# Autodesk Inventor assembly: Assembly_v1
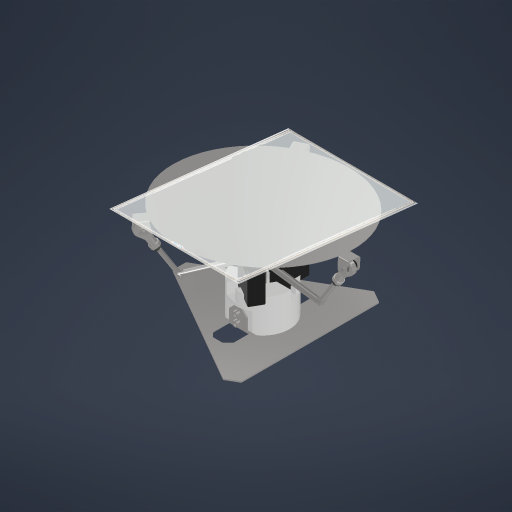
[picture p0: Inventor's stored thumbnail of the model, 512x512]
Saved by Autodesk Inventor 2023 (Build 270158000, 158)
## iProperties
Created: 2023-02-24
Part Number: Assembly_v1
Document SubType Name: Assembly
Designer: roota
Mass: 2034.34 g
Surface Area: 3097.58 cm^2
Volume: 420.227 cm^3
Density: 4.84106 g/cm^3
Author: roota
## Documents named in this file (20)
- D:\GitHub\NTUST-Mechanical-Design\Ball stabilization mechanism\3D CAD files\Mechanical Part CAD files\Assemblies\Assembly_v1.iam
- D:\GitHub\NTUST-Mechanical-Design\Ball stabilization mechanism\3D CAD files\Mechanical Part CAD files\Static Mechanisms\BalancePlate.ipt
- D:\GitHub\NTUST-Mechanical-Design\Ball stabilization mechanism\3D CAD files\Mechanical Part CAD files\Static Mechanisms\BasePlate.ipt
- D:\GitHub\NTUST-Mechanical-Design\Ball stabilization mechanism\3D CAD files\Mechanical Part CAD files\Static Mechanisms\BaseSupport.ipt
- C:\Users\roota\Documents\Inventor\Content Center Files\R2023\en-US\JIS B 2804 E\_JIS B 2804 E - 5 - 6.ipt
- D:\GitHub\NTUST-Mechanical-Design\Ball stabilization mechanism\3D CAD files\Mechanical Part CAD files\Static Mechanisms\rod pin.ipt
- D:\GitHub\NTUST-Mechanical-Design\Ball stabilization mechanism\3D CAD files\Mechanical Part CAD files\Static Mechanisms\4mm spacer.ipt
- D:\GitHub\NTUST-Mechanical-Design\Ball stabilization mechanism\3D CAD files\Mechanical Part CAD files\Hardware Parts\SELF-LUBRIFICATING ROD END\Ball_6mm.ipt
- D:\GitHub\NTUST-Mechanical-Design\Ball stabilization mechanism\3D CAD files\Mechanical Part CAD files\Hardware Parts\SELF-LUBRIFICATING ROD END\End_6mm.ipt
- D:\GitHub\NTUST-Mechanical-Design\Ball stabilization mechanism\3D CAD files\Mechanical Part CAD files\Hardware Parts\M6x1_THREADED_ROD.ipt
- D:\GitHub\NTUST-Mechanical-Design\Ball stabilization mechanism\3D CAD files\Mechanical Part CAD files\Hardware Parts\5mm Bushing.ipt
- D:\GitHub\NTUST-Mechanical-Design\Ball stabilization mechanism\3D CAD files\Mechanical Part CAD files\Dynamic Mechanisms\Servo_Strut.ipt
- C:\Users\roota\Documents\Inventor\Content Center Files\R2023\en-US\ISO 4762(2)\ISO 4762 - M3 x 8ISO.ipt
- D:\GitHub\NTUST-Mechanical-Design\Ball stabilization mechanism\3D CAD files\Mechanical Part CAD files\Hardware Parts\12_1_INCH_TOUCHSCREEN\12inch Touchscreen.ipt
- C:\Users\roota\Documents\Inventor\Content Center Files\R2023\en-US\ISO 4036(2)\ISO 4036 - M6(2).ipt
- C:\Users\roota\Documents\Inventor\Content Center Files\R2023\en-US\ISO 4762(2)\ISO 4762 - M5 x 8ISO.ipt
- D:\GitHub\NTUST-Mechanical-Design\Ball stabilization mechanism\3D CAD files\Electrical Hardware CAD files\SERVO\LDX-335MG_Servo_15kg_cm.ipt
- C:\Users\roota\Documents\Inventor\Content Center Files\R2023\en-US\BS EN ISO 4026\BS EN ISO 4168 - M3 x 6(2).ipt
- D:\GitHub\NTUST-Mechanical-Design\Ball stabilization mechanism\3D CAD files\Mechanical Part CAD files\Static Mechanisms\ServoCap.ipt
- C:\Users\roota\Documents\Inventor\Content Center Files\R2023\en-US\ISO 10642(1)\ISO 10642 - M8 x  60.ipt
## Components (58 placed, 19 different names)
1. BalancePlate:1 — Mate:6, Mate:9, Mate:10, Mate:11, Mate:12, Mate:60, Mate:61, Mate:62, Mate:64, Mate:65, Mate:67, Mate:68, Flush:1, Flush:2, Mate:70, Mate:71, Mate:72, Mate:73, Mate:74, Mate:75, Mate:76, Mate:77, Mate:78, Mate:79, Mate:80, Mate:81, Mate:91, Mate:101
2. BasePlate:1 — Mate:1, Mate:2, Mate:3, Insert:4, Insert:5, Insert:6, Insert:7
3. BaseSupport:1 — Mate:1, Mate:2, Mate:3, Mate:87, Mate:88, Mate:103, Mate:104, Mate:106, Mate:107, Mate:114, Mate:115, Mate:116, Mate:117, Mate:119, Mate:120, Mate:126
4. JIS B 2804 E 5:5 — Mate:5, Mate:8, Mate:10
5. JIS B 2804 E 5:6 — Mate:4, Mate:7
6. rod pin:3 — Mate:4, Mate:5, Mate:6, Mate:7, Mate:8, Mate:9, Mate:13, Mate:14, Mate:15
7. 4mm spacer:1 — Mate:12, Mate:13
8. 4mm spacer:2 — Mate:11, Mate:14, Mate:16
9. Ball_6mm:1 — Mate:15, Mate:16, Mate:17
10. End_6mm:1 — Mate:17, Mate:18, Mate:19, Angle:1, Insert:1
11. M6x1_THREADED_ROD:1 — Mate:18, Mate:19, Mate:20, Mate:23, Angle:1
12. 5mm Bushing:1 — Mate:20, Mate:21, Mate:22, Mate:24
13. Servo_Strut:1 — Mate:21, Mate:22, Mate:23, Mate:25, Mate:85, Mate:86
14. ISO 4762 M3 x 8:1 — Mate:24, Mate:25
15. ISO 4036 M6:1 — Insert:1
16. 12inch Touchscreen:1 — Mate:68, Flush:1, Flush:2
17. JIS B 2804 E 5:7 — Mate:72, Mate:73, Mate:82
18. JIS B 2804 E 5:8 — Mate:62, Mate:74, Mate:75
19. 4mm spacer:5 — Mate:60, Mate:61
20. Ball_6mm:2 — Mate:34, Mate:78, Mate:102
21. End_6mm:2 — Mate:34, Angle:2, Mate:35, Mate:36, Insert:2
22. M6x1_THREADED_ROD:2 — Angle:2, Mate:35, Mate:36, Mate:37, Mate:99
23. 5mm Bushing:2 — Mate:37, Mate:42, Mate:96, Mate:97
24. ISO 4762 M3 x 8:2 — Mate:42, Mate:98
25. ISO 4036 M6:2 — Insert:2
26. JIS B 2804 E 5:10 — Mate:67, Mate:76, Mate:77, Mate:83
27. 4mm spacer:6 — Mate:50, Mate:64, Mate:65
28. Ball_6mm:3 — Mate:50, Mate:51, Mate:79
29. End_6mm:3 — Mate:51, Mate:52, Mate:53, Angle:3, Insert:3
30. M6x1_THREADED_ROD:3 — Mate:52, Mate:53, Angle:3, Mate:54, Mate:95
31. 5mm Bushing:3 — Mate:54, Mate:58, Mate:92, Mate:93
32. ISO 4762 M3 x 8:3 — Mate:58, Mate:94
33. ISO 4036 M6:3 — Insert:3
34. ISO 4762 M5 x 8:1 — Insert:4
35. ISO 4762 M5 x 8:2 — Insert:5
36. ISO 4762 M5 x 8:3 — Insert:6, Mate:126
37. ISO 4762 M5 x 8:4 — Insert:7
38. JIS B 2804 E 5:12 — Mate:70, Mate:71
39. rod pin:4 — Mate:81, Mate:82, Mate:100
40. rod pin:5 — Mate:80, Mate:83, Mate:90
41. LDX-335MG_Servo_15kg_cm:1 — Mate:85, Mate:86, Mate:87, Mate:88, Mate:116, Mate:122, Insert:10, Insert:11
42. 4mm spacer:3 — Mate:90, Mate:91
43. Servo_Strut:2 — Mate:92, Mate:93, Mate:94, Mate:95, Mate:110, Mate:111
44. Servo_Strut:3 — Mate:96, Mate:97, Mate:98, Mate:99, Mate:112, Mate:113
45. 4mm spacer:4 — Mate:100, Mate:101, Mate:102
46. LDX-335MG_Servo_15kg_cm:2 — Mate:103, Mate:106, Mate:110, Mate:111, Mate:114, Mate:121, Insert:12, Insert:13
47. LDX-335MG_Servo_15kg_cm:3 — Mate:104, Mate:107, Mate:112, Mate:113, Mate:115, Mate:118, Insert:8, Insert:9
48. BS EN ISO 4026 - Metric M3 x 6:1 — Mate:117, Mate:118
49. BS EN ISO 4026 - Metric M3 x 6:2 — Mate:120, Mate:121
50. BS EN ISO 4026 - Metric M3 x 6:3 — Mate:119, Mate:122
51. ISO 10642 M8x60:1
52. ServoCap:1
53. ISO 4762 M5 x 8:7 — Insert:8
54. ISO 4762 M5 x 8:8 — Insert:9
55. ISO 4762 M5 x 8:9 — Insert:10
56. ISO 4762 M5 x 8:10 — Insert:11
57. ISO 4762 M5 x 8:11 — Insert:12
58. ISO 4762 M5 x 8:12 — Insert:13
## Relationships (110: Mate 92, Insert 13, Angle 3, Flush 2)
- Mate:1: BasePlate:1 ↔ BaseSupport:1
- Mate:2: BasePlate:1 ↔ BaseSupport:1
- Mate:3: BasePlate:1 ↔ BaseSupport:1
- Mate:4: JIS B 2804 E 5:6 ↔ rod pin:3
- Mate:5: JIS B 2804 E 5:5 ↔ rod pin:3
- Mate:6: BalancePlate:1 ↔ rod pin:3
- Mate:7: JIS B 2804 E 5:6 ↔ rod pin:3
- Mate:8: JIS B 2804 E 5:5 ↔ rod pin:3
- Mate:9: BalancePlate:1 ↔ rod pin:3
- Mate:10: BalancePlate:1 ↔ JIS B 2804 E 5:5
- Mate:11: BalancePlate:1 ↔ 4mm spacer:2
- Mate:12: BalancePlate:1 ↔ 4mm spacer:1
- Mate:13: rod pin:3 ↔ 4mm spacer:1
- Mate:14: rod pin:3 ↔ 4mm spacer:2
- Mate:15: rod pin:3 ↔ Ball_6mm:1
- Mate:16: 4mm spacer:2 ↔ Ball_6mm:1
- Mate:17: Ball_6mm:1 ↔ End_6mm:1
- Mate:18: End_6mm:1 ↔ M6x1_THREADED_ROD:1
- Mate:19 (-8 mm): End_6mm:1 ↔ M6x1_THREADED_ROD:1
- Mate:20: M6x1_THREADED_ROD:1 ↔ 5mm Bushing:1
- Mate:21: 5mm Bushing:1 ↔ Servo_Strut:1
- Mate:22: 5mm Bushing:1 ↔ Servo_Strut:1
- Mate:23: M6x1_THREADED_ROD:1 ↔ Servo_Strut:1
- Angle:1 (0 deg): End_6mm:1 ↔ M6x1_THREADED_ROD:1
- Mate:24: 5mm Bushing:1 ↔ ISO 4762 M3 x 8:1
- Mate:25: Servo_Strut:1 ↔ ISO 4762 M3 x 8:1
- Insert:1: End_6mm:1 ↔ ISO 4036 M6:1
- Mate:34: Ball_6mm:2 ↔ End_6mm:2
- Angle:2 (0 deg): End_6mm:2 ↔ M6x1_THREADED_ROD:2
- Mate:35 (-8 mm): End_6mm:2 ↔ M6x1_THREADED_ROD:2
- Mate:36: End_6mm:2 ↔ M6x1_THREADED_ROD:2
- Mate:37: M6x1_THREADED_ROD:2 ↔ 5mm Bushing:2
- Mate:42: 5mm Bushing:2 ↔ ISO 4762 M3 x 8:2
- Insert:2: End_6mm:2 ↔ ISO 4036 M6:2
- Mate:50: 4mm spacer:6 ↔ Ball_6mm:3
- Mate:51: Ball_6mm:3 ↔ End_6mm:3
- Mate:52: End_6mm:3 ↔ M6x1_THREADED_ROD:3
- Mate:53 (-8 mm): End_6mm:3 ↔ M6x1_THREADED_ROD:3
- Angle:3 (0 deg): End_6mm:3 ↔ M6x1_THREADED_ROD:3
- Mate:54: M6x1_THREADED_ROD:3 ↔ 5mm Bushing:3
- Mate:58: 5mm Bushing:3 ↔ ISO 4762 M3 x 8:3
- Insert:3: End_6mm:3 ↔ ISO 4036 M6:3
- Mate:60: BalancePlate:1 ↔ 4mm spacer:5
- Mate:61: BalancePlate:1 ↔ 4mm spacer:5
- Mate:62: BalancePlate:1 ↔ JIS B 2804 E 5:8
- Mate:64: BalancePlate:1 ↔ 4mm spacer:6
- Mate:65: BalancePlate:1 ↔ 4mm spacer:6
- Mate:67: BalancePlate:1 ↔ JIS B 2804 E 5:10
- Insert:4: BasePlate:1 ↔ ISO 4762 M5 x 8:1
- Insert:5: BasePlate:1 ↔ ISO 4762 M5 x 8:2
- Insert:6: BasePlate:1 ↔ ISO 4762 M5 x 8:3
- Insert:7: BasePlate:1 ↔ ISO 4762 M5 x 8:4
- Mate:68: BalancePlate:1 ↔ 12inch Touchscreen:1
- Flush:1 (-40 mm): BalancePlate:1 ↔ 12inch Touchscreen:1
- Flush:2 (120 mm): BalancePlate:1 ↔ 12inch Touchscreen:1
- Mate:70: BalancePlate:1 ↔ JIS B 2804 E 5:12
- Mate:71: BalancePlate:1 ↔ JIS B 2804 E 5:12
- Mate:72: BalancePlate:1 ↔ JIS B 2804 E 5:7
- Mate:73: BalancePlate:1 ↔ JIS B 2804 E 5:7
- Mate:74: BalancePlate:1 ↔ JIS B 2804 E 5:8
- Mate:75: BalancePlate:1 ↔ JIS B 2804 E 5:8
- Mate:76: BalancePlate:1 ↔ JIS B 2804 E 5:10
- Mate:77: BalancePlate:1 ↔ JIS B 2804 E 5:10
- Mate:78: BalancePlate:1 ↔ Ball_6mm:2
- Mate:79: BalancePlate:1 ↔ Ball_6mm:3
- Mate:80: BalancePlate:1 ↔ rod pin:5
- Mate:81: BalancePlate:1 ↔ rod pin:4
- Mate:82: JIS B 2804 E 5:7 ↔ rod pin:4
- Mate:83: JIS B 2804 E 5:10 ↔ rod pin:5
- Mate:85: Servo_Strut:1 ↔ LDX-335MG_Servo_15kg_cm:1
- Mate:86: Servo_Strut:1 ↔ LDX-335MG_Servo_15kg_cm:1
- Mate:87: BaseSupport:1 ↔ LDX-335MG_Servo_15kg_cm:1
- Mate:88: BaseSupport:1 ↔ LDX-335MG_Servo_15kg_cm:1
- Mate:90: rod pin:5 ↔ 4mm spacer:3
- Mate:91: BalancePlate:1 ↔ 4mm spacer:3
- Mate:92: 5mm Bushing:3 ↔ Servo_Strut:2
- Mate:93: 5mm Bushing:3 ↔ Servo_Strut:2
- Mate:94: ISO 4762 M3 x 8:3 ↔ Servo_Strut:2
- Mate:95: M6x1_THREADED_ROD:3 ↔ Servo_Strut:2
- Mate:96: 5mm Bushing:2 ↔ Servo_Strut:3
- Mate:97: 5mm Bushing:2 ↔ Servo_Strut:3
- Mate:98: ISO 4762 M3 x 8:2 ↔ Servo_Strut:3
- Mate:99: M6x1_THREADED_ROD:2 ↔ Servo_Strut:3
- Mate:100: rod pin:4 ↔ 4mm spacer:4
- Mate:101: BalancePlate:1 ↔ 4mm spacer:4
- Mate:102: Ball_6mm:2 ↔ 4mm spacer:4
- Mate:103: BaseSupport:1 ↔ LDX-335MG_Servo_15kg_cm:2
- Mate:104: BaseSupport:1 ↔ LDX-335MG_Servo_15kg_cm:3
- Mate:106: BaseSupport:1 ↔ LDX-335MG_Servo_15kg_cm:2
- Mate:107: BaseSupport:1 ↔ LDX-335MG_Servo_15kg_cm:3
- Mate:110: Servo_Strut:2 ↔ LDX-335MG_Servo_15kg_cm:2
- Mate:111: Servo_Strut:2 ↔ LDX-335MG_Servo_15kg_cm:2
- Mate:112: Servo_Strut:3 ↔ LDX-335MG_Servo_15kg_cm:3
- Mate:113: Servo_Strut:3 ↔ LDX-335MG_Servo_15kg_cm:3
- Mate:114: BaseSupport:1 ↔ LDX-335MG_Servo_15kg_cm:2
- Mate:115: BaseSupport:1 ↔ LDX-335MG_Servo_15kg_cm:3
- Mate:116: BaseSupport:1 ↔ LDX-335MG_Servo_15kg_cm:1
- Mate:117: BaseSupport:1 ↔ BS EN ISO 4026 - Metric M3 x 6:1
- Mate:118: LDX-335MG_Servo_15kg_cm:3 ↔ BS EN ISO 4026 - Metric M3 x 6:1
- Mate:119: BaseSupport:1 ↔ BS EN ISO 4026 - Metric M3 x 6:3
- Mate:120: BaseSupport:1 ↔ BS EN ISO 4026 - Metric M3 x 6:2
- Mate:121: LDX-335MG_Servo_15kg_cm:2 ↔ BS EN ISO 4026 - Metric M3 x 6:2
- Mate:122: LDX-335MG_Servo_15kg_cm:1 ↔ BS EN ISO 4026 - Metric M3 x 6:3
- Mate:126: BaseSupport:1 ↔ ISO 4762 M5 x 8:3
- Insert:8: LDX-335MG_Servo_15kg_cm:3 ↔ ISO 4762 M5 x 8:7
- Insert:9: LDX-335MG_Servo_15kg_cm:3 ↔ ISO 4762 M5 x 8:8
- Insert:10: LDX-335MG_Servo_15kg_cm:1 ↔ ISO 4762 M5 x 8:9
- Insert:11: LDX-335MG_Servo_15kg_cm:1 ↔ ISO 4762 M5 x 8:10
- Insert:12: LDX-335MG_Servo_15kg_cm:2 ↔ ISO 4762 M5 x 8:11
- Insert:13: LDX-335MG_Servo_15kg_cm:2 ↔ ISO 4762 M5 x 8:12
## Named parameters: SERVO_DIAM = 0 mm, J1 = 0 mm, J2 = 0 mm, J3 = 0 mm
